# Autodesk Inventor assembly: Tire_v6
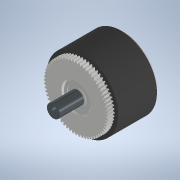
[picture p0: Inventor's stored thumbnail of the model, 180x180]
Saved by Autodesk Inventor 2022 (Build 260153000, 153)
## iProperties
Created: 2022-07-22
Part Number: Tire_v6
Document SubType Name: Assembly
Designer: Yazawa
Author: Yazawa
## Documents named in this file (5)
- C:\Users\Yazawa\Documents\GitHub\murakumo\inventor\Tire_v6.iam
- C:\Users\Yazawa\Documents\GitHub\murakumo\inventor\wheel_v6.ipt
- C:\Users\Yazawa\Documents\GitHub\murakumo\inventor\Tire.ipt
- C:\Users\Yazawa\Documents\GitHub\murakumo\inventor\FL674ZZ.ipt
- C:\Users\Yazawa\Documents\GitHub\murakumo\inventor\shaft.ipt
## Components (5 placed, 4 different names)
1. wheel_v6:1 — メイト:1, メイト:2, メイト:3, メイト:5, メイト:6, メイト:8
2. Tire:1 — メイト:1, メイト:2
3. FL674ZZ:1 — メイト:3, メイト:8
4. FL674ZZ:2 — メイト:5, メイト:6, メイト:7, フラッシュ:1
5. shaft:1 — メイト:7, フラッシュ:1
## Relationships (8: Mate 7, Flush 1)
- メイト:1 [Mate]: wheel_v6:1 ↔ Tire:1
- メイト:2 [Mate]: wheel_v6:1 ↔ Tire:1
- メイト:3 [Mate]: wheel_v6:1 ↔ FL674ZZ:1
- メイト:5 [Mate]: wheel_v6:1 ↔ FL674ZZ:2
- メイト:6 [Mate]: wheel_v6:1 ↔ FL674ZZ:2
- メイト:7 [Mate]: FL674ZZ:2 ↔ shaft:1
- フラッシュ:1 [Flush]: FL674ZZ:2 ↔ shaft:1
- メイト:8 [Mate]: wheel_v6:1 ↔ FL674ZZ:1
